# Autodesk Inventor assembly: 000_SU22_EncorderUnit_sn_MIR
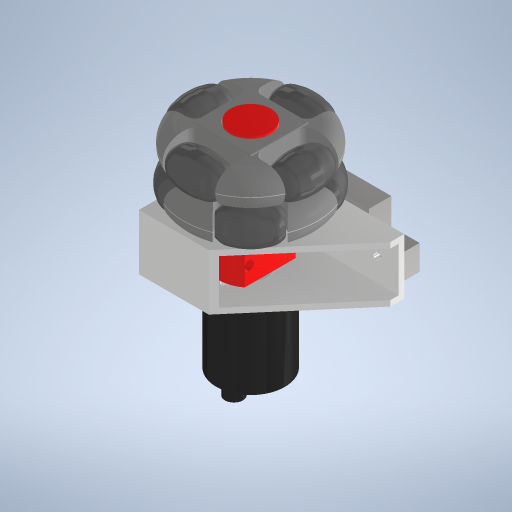
[picture p0: Inventor's stored thumbnail of the model, 512x512]
Saved by Autodesk Inventor 2023 (Build 270158000, 158)
## iProperties
Created: 2022-06-28
Part Number: 000_SU22_EncorderUnit_sn_MIR
Document SubType Name: Assembly
Designer: 中島 青蔵
Author: 中島 青蔵
## Documents named in this file (9)
- C:\Users\blueh\OneDrive - Kyushu University\夏ロボ_sn\000_SU22_EncorderUnit_sn_MIR.iam
- C:\Users\blueh\OneDrive - Kyushu University\夏ロボ_sn\ROTACASTER_48_KH_MIR.iam
- C:\Users\blueh\OneDrive - Kyushu University\夏ロボ_sn\encoder v3_MIR.ipt
- C:\Users\blueh\OneDrive - Kyushu University\夏ロボ_sn\SU22_3DP_EncorderUnit_Bar_sn_MIR.ipt
- C:\Users\blueh\OneDrive - Kyushu University\夏ロボ_sn\SU22_SQP_20_40_EU_sn_MIR.ipt
- C:\Users\blueh\OneDrive - Kyushu University\夏ロボ_sn\SU22_Bearing_8_12_13.6_sn_MIR.ipt
- C:\Users\blueh\OneDrive - Kyushu University\夏ロボ_sn\SU22_3DP_EU_Sub_sn_MIR.ipt
- C:\Users\blueh\OneDrive - Kyushu University\夏ロボ_sn\SU22_Slider_55_sn_MIR.ipt
- C:\Users\blueh\OneDrive - Kyushu University\夏ロボ_sn\SU22_Slider_Box_sn_MIR.ipt
## Components (8 placed, 8 different names)
1. ROTACASTER_48_KH_MIR:1 [sub-assembly] — 挿入:1
2. encoder v3_MIR:1 — 角度:1, 挿入:5, 挿入:4
3. SU22_3DP_EncorderUnit_Bar_sn_MIR:1 — 挿入:1, 角度:1, 挿入:3, 角度:2, 挿入:6
4. SU22_SQP_20_40_EU_sn_MIR:1 — 挿入:5, 挿入:4, 挿入:2, 挿入:8, 挿入:7
5. SU22_Bearing_8_12_13.6_sn_MIR:1 — 挿入:3, 挿入:2
6. SU22_3DP_EU_Sub_sn_MIR:1 — 角度:2, 挿入:6
7. SU22_Slider_55_sn_MIR:1 — 挿入:8, 挿入:7, メイト:2, メイト:1
8. SU22_Slider_Box_sn_MIR:1 — メイト:2, メイト:1
## Relationships (12: Insert 8, Angle 2, Mate 2)
- 挿入:1 [Insert]: ROTACASTER_48_KH_MIR:1 ↔ SU22_3DP_EncorderUnit_Bar_sn_MIR:1
- 角度:1 [Angle] (0 deg): encoder v3_MIR:1 ↔ SU22_3DP_EncorderUnit_Bar_sn_MIR:1
- 挿入:5 [Insert]: encoder v3_MIR:1 ↔ SU22_SQP_20_40_EU_sn_MIR:1
- 挿入:4 [Insert]: encoder v3_MIR:1 ↔ SU22_SQP_20_40_EU_sn_MIR:1
- 挿入:3 [Insert]: SU22_3DP_EncorderUnit_Bar_sn_MIR:1 ↔ SU22_Bearing_8_12_13.6_sn_MIR:1
- 挿入:2 [Insert]: SU22_SQP_20_40_EU_sn_MIR:1 ↔ SU22_Bearing_8_12_13.6_sn_MIR:1
- 角度:2 [Angle] (0 deg): SU22_3DP_EncorderUnit_Bar_sn_MIR:1 ↔ SU22_3DP_EU_Sub_sn_MIR:1
- 挿入:6 [Insert]: SU22_3DP_EncorderUnit_Bar_sn_MIR:1 ↔ SU22_3DP_EU_Sub_sn_MIR:1
- 挿入:8 [Insert]: SU22_SQP_20_40_EU_sn_MIR:1 ↔ SU22_Slider_55_sn_MIR:1
- 挿入:7 [Insert]: SU22_SQP_20_40_EU_sn_MIR:1 ↔ SU22_Slider_55_sn_MIR:1
- メイト:2 [Mate]: SU22_Slider_55_sn_MIR:1 ↔ SU22_Slider_Box_sn_MIR:1
- メイト:1 [Mate]: SU22_Slider_55_sn_MIR:1 ↔ SU22_Slider_Box_sn_MIR:1
